# Autodesk Inventor assembly: Infill3DExtruderRightMirrored
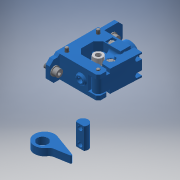
[picture p0: Inventor's stored thumbnail of the model, 180x180]
Saved by Autodesk Inventor 2016 (Build 200138000, 138)
## iProperties
Created: 2015-04-27
Part Number: Infill3DExtruderRightMirrored
Document SubType Name: Assembly
Designer: Jack
Author: Jack
## Documents named in this file (13)
- C:\Users\Jack\ownCloud\Projects\CrossBot\InventorModel\Extruder\Infill3DExtruder\Infill3DExtruderLeft.iam
- C:\Users\Jack\ownCloud\Projects\CrossBot\InventorModel\Extruder\Infill3DExtruder\Infill3DBodyLeft.ipt
- C:\Users\Jack\ownCloud\Projects\CrossBot\InventorModel\Electronics\Motors\StepperMotorNema17x60mm.ipt
- C:\Users\Jack\ownCloud\Projects\CrossBot\InventorModel\Hardware\Extruder\DriveGearMK8.ipt
- C:\Users\Jack\ownCloud\Projects\CrossBot\InventorModel\Extruder\Infill3DExtruder\Infill3DIdlerLeft.ipt
- C:\Users\Jack\ownCloud\Projects\CrossBot\InventorModel\Hardware\Bearing\BearingRadialBall\BearingRadialBall624zz.ipt
- C:\Users\Jack\ownCloud\Projects\CrossBot\InventorModel\Hardware\Nuts\Nut4.ipt
- C:\Users\Jack\ownCloud\Projects\CrossBot\InventorModel\Hardware\Bolts\SHCS\SHCS4\SHCS4x16.ipt
- C:\Users\Jack\ownCloud\Projects\CrossBot\InventorModel\Hardware\BoltWashers\BoltWasher4\BoltWasher4x10.iam
- C:\Users\Jack\ownCloud\Projects\CrossBot\InventorModel\Hardware\Bolts\SHCS\SHCS3\SHCS3x10.ipt
- C:\Users\Jack\ownCloud\Projects\CrossBot\InventorModel\Hardware\Bolts\SHCS\SHCS3\SHCS3x20.ipt
- C:\Users\Jack\ownCloud\Projects\CrossBot\InventorModel\Extruder\Infill3DExtruder\Infill3DExtruderTensionCam.ipt
- C:\Users\Jack\ownCloud\Projects\CrossBot\InventorModel\Extruder\Infill3DExtruder\Infill3DExtruderTensionDowel.ipt
## Components (16 placed, 12 different names)
1. Infill3DBodyLeft:1 — Mate:6, Mate:2, Mate:1, Mate:8, Mate:7, Angle:3, Mate:18, Mate:20, Mate:24, Mate:21, Mate:23, Mate:22, Mate:24, Mate:25, Mate:26, Mate:27, Mate:28, Mate:29, Angle:4, Mate:30
2. StepperMotorNema17x60mm:1 — Mate:6, Mate:2, Mate:1, Mate:5, Mate:4
3. DriveGearMK8:1 — Mate:5, Mate:4
4. Infill3DIdlerLeft:1 — Mate:8, Mate:7, Mate:10, Mate:9, Mate:11, Mate:14, Mate:13, Angle:5, Mate:31
5. BearingRadialBall624zz:1 — Mate:10, Mate:9
6. Nut4:1 — Mate:11, Angle:5, Mate:31
7. SHCS4x16:1 — Mate:14, Mate:13
8. Nut4:2 — Angle:3, Mate:18
9. Nut4:3 — Mate:20, Angle:4, Mate:30
10. BoltWasher4x10:1 [sub-assembly] — Mate:24, Mate:21
11. BoltWasher4x10:2 [sub-assembly] — Mate:23, Mate:22
12. SHCS3x10:1 — Mate:24, Mate:27
13. SHCS3x10:2 — Mate:25, Mate:26
14. SHCS3x20:1 — Mate:28, Mate:29
15. Infill3DExtruderTensionCam:1
16. Infill3DExtruderTensionDowel:1
## Relationships (29: Mate 26, Angle 3)
- Mate:6: Infill3DBodyLeft:1 ↔ StepperMotorNema17x60mm:1
- Mate:2: Infill3DBodyLeft:1 ↔ StepperMotorNema17x60mm:1
- Mate:1: Infill3DBodyLeft:1 ↔ StepperMotorNema17x60mm:1
- Mate:5 (1 mm): StepperMotorNema17x60mm:1 ↔ DriveGearMK8:1
- Mate:4: StepperMotorNema17x60mm:1 ↔ DriveGearMK8:1
- Mate:8 (0.2 mm): Infill3DBodyLeft:1 ↔ Infill3DIdlerLeft:1
- Mate:7: Infill3DBodyLeft:1 ↔ Infill3DIdlerLeft:1
- Mate:10: Infill3DIdlerLeft:1 ↔ BearingRadialBall624zz:1
- Mate:9: Infill3DIdlerLeft:1 ↔ BearingRadialBall624zz:1
- Mate:11: Infill3DIdlerLeft:1 ↔ Nut4:1
- Mate:14: Infill3DIdlerLeft:1 ↔ SHCS4x16:1
- Mate:13: Infill3DIdlerLeft:1 ↔ SHCS4x16:1
- Angle:3 (0 deg): Infill3DBodyLeft:1 ↔ Nut4:2
- Mate:18: Infill3DBodyLeft:1 ↔ Nut4:2
- Mate:20: Infill3DBodyLeft:1 ↔ Nut4:3
- Mate:24: Infill3DBodyLeft:1 ↔ BoltWasher4x10:1
- Mate:21: Infill3DBodyLeft:1 ↔ BoltWasher4x10:1
- Mate:23: Infill3DBodyLeft:1 ↔ BoltWasher4x10:2
- Mate:22: Infill3DBodyLeft:1 ↔ BoltWasher4x10:2
- Mate:24: Infill3DBodyLeft:1 ↔ SHCS3x10:1
- Mate:25: Infill3DBodyLeft:1 ↔ SHCS3x10:2
- Mate:26: Infill3DBodyLeft:1 ↔ SHCS3x10:2
- Mate:27: Infill3DBodyLeft:1 ↔ SHCS3x10:1
- Mate:28: Infill3DBodyLeft:1 ↔ SHCS3x20:1
- Mate:29: Infill3DBodyLeft:1 ↔ SHCS3x20:1
- Angle:4 (0 deg): Infill3DBodyLeft:1 ↔ Nut4:3
- Mate:30: Infill3DBodyLeft:1 ↔ Nut4:3
- Angle:5 (0 deg): Infill3DIdlerLeft:1 ↔ Nut4:1
- Mate:31: Infill3DIdlerLeft:1 ↔ Nut4:1
